# Autodesk Inventor assembly: TUBING NOTCHER DIE
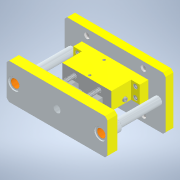
[picture p0: Inventor's stored thumbnail of the model, 180x180]
Saved by Autodesk Inventor 2021 (Build 250183000, 183)
## iProperties
Company: Unknown
Created: 2021-06-05
Part Number: TUBING NOTCHER DIE
Description: Unknown
Document SubType Name: Assembly
Designer: Nelson
Sending System: Unknown
Preprocessor: PSStep 14.0
Title: D:/TRABAJO EN SOLID ST4/PROYECTOS  SOLID ST4/TROQUEL RECORTAR EXTREMO TUBO GT/IMAGENES/TUBING NOTCHER DIE.stp
Author: Unknown
Revision Number: NONE
## Documents named in this file (27)
- D:\Nelson\Documentos\Inventor\PrensaHidraulica_Automatizada\TUBING NOTCHER DIE.iam
- D:\Nelson\Documentos\Inventor\PrensaHidraulica_Automatizada\SOPORTE.ipt
- D:\Nelson\Documentos\Inventor\PrensaHidraulica_Automatizada\EMPUJADOR.ipt
- D:\Nelson\Documentos\Inventor\PrensaHidraulica_Automatizada\LEVA_102.ipt
- D:\Nelson\Documentos\Inventor\PrensaHidraulica_Automatizada\LEVA_104.ipt
- D:\Nelson\Documentos\Inventor\PrensaHidraulica_Automatizada\LEVA_MATRIZ_106.ipt
- D:\Nelson\Documentos\Inventor\PrensaHidraulica_Automatizada\PUNZON.ipt
- D:\Nelson\Documentos\Inventor\PrensaHidraulica_Automatizada\PORTA_MATRIZ.ipt
- D:\Nelson\Documentos\Inventor\PrensaHidraulica_Automatizada\MATRIZ.ipt
- D:\Nelson\Documentos\Inventor\PrensaHidraulica_Automatizada\SUPLEMENTO MATRIZ.ipt
- D:\Nelson\Documentos\Inventor\PrensaHidraulica_Automatizada\GUIA.ipt
- D:\Nelson\Documentos\Inventor\PrensaHidraulica_Automatizada\RESORTE COMPRESION.ipt
- D:\Nelson\Documentos\Inventor\PrensaHidraulica_Automatizada\PLACA BASE.ipt
- D:\Nelson\Documentos\Inventor\PrensaHidraulica_Automatizada\PLACA SUPERIOR.ipt
- D:\Nelson\Documentos\Inventor\PrensaHidraulica_Automatizada\CASQUILLO 2051_32_032_060_10 FIBRO.ipt
- D:\Nelson\Documentos\Inventor\PrensaHidraulica_Automatizada\_202.21.032.200.10(ET).ipt
- D:\Nelson\Documentos\Inventor\PrensaHidraulica_Automatizada\_202.41.01732.ipt
- D:\Nelson\Documentos\Inventor\PrensaHidraulica_Automatizada\_2192.10.16.040.ipt
- D:\Nelson\Documentos\Inventor\PrensaHidraulica_Automatizada\LIMITADOR CARRERA.ipt
- D:\Nelson\Documentos\Inventor\PrensaHidraulica_Automatizada\PRIS DIN_915-M8x20.ipt
- D:\Nelson\Documentos\Inventor\PrensaHidraulica_Automatizada\DIN 7_8m6x30.ipt
- D:\Nelson\Documentos\Inventor\PrensaHidraulica_Automatizada\DIN 7_10m6x60.ipt
- D:\Nelson\Documentos\Inventor\PrensaHidraulica_Automatizada\PASADOR DIN1480 8_x_50_st.ipt
- D:\Nelson\Documentos\Inventor\PrensaHidraulica_Automatizada\ALLEN DIN 912 10x30.ipt
- D:\Nelson\Documentos\Inventor\PrensaHidraulica_Automatizada\ALLEN DIN 012-M10x40.ipt
- D:\Nelson\Documentos\Inventor\PrensaHidraulica_Automatizada\ALLEN DIN 912 - M8x25.ipt
- D:\Nelson\Documentos\Inventor\PrensaHidraulica_Automatizada\ALLEN DIN 912 10x60.ipt
## Components (43 placed, 26 different names)
1. SOPORTE
2. EMPUJADOR
3. LEVA_102
4. LEVA_104
5. LEVA_MATRIZ_106 — Mate:1
6. PORTA_MATRIZ
7. MATRIZ
8. SUPLEMENTO MATRIZ
9. GUIA
10. GUIA:1
11. RESORTE COMPRESION
12. RESORTE COMPRESION:1
13. PLACA BASE
14. PLACA SUPERIOR
15. CASQUILLO 2051_32_032_060_10 FIBRO
16. CASQUILLO 2051_32_032_060_10 FIBRO:1
17. _202.21.032.200.10(ET)
18. _202.21.032.200.10(ET):1
19. _202.41.01732
20. _202.41.01732:1
21. _2192.10.16.040
22. _2192.10.16.040:1
23. LIMITADOR CARRERA
24. LIMITADOR CARRERA:1
25. PRIS DIN_915-M8x20
26. PRIS DIN_915-M8x20:1
27. DIN 7_8m6x30
28. DIN 7_8m6x30:1
29. DIN 7_10m6x60
30. DIN 7_10m6x60:1
31. PASADOR DIN1480 8_x_50_st — Mate:2
32. ALLEN DIN 912 10x30
33. ALLEN DIN 912 10x30:1
34. ALLEN DIN 012-M10x40
35. ALLEN DIN 012-M10x40:1
36. ALLEN DIN 012-M10x40:2
37. ALLEN DIN 912 - M8x25
38. ALLEN DIN 912 - M8x25:1
39. ALLEN DIN 912 10x60
40. ALLEN DIN 912 10x60:1
41. ALLEN DIN 912 10x60:2
42. ALLEN DIN 912 10x60:3
43. PUNZON:2 — Mate:1, Mate:2
## Relationships (2: Mate 2)
- Mate:1: LEVA_MATRIZ_106 ↔ PUNZON:2
- Mate:2: PASADOR DIN1480 8_x_50_st ↔ PUNZON:2
